# Autodesk Inventor assembly: Prototype2
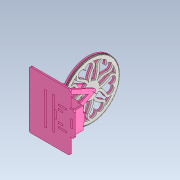
[picture p0: Inventor's stored thumbnail of the model, 180x180]
Saved by Autodesk Inventor 2021 (Build 250183000, 183)
## iProperties
Created: 2021-08-31
Part Number: Prototype2
Document SubType Name: Assembly
Designer: digge
Author: digge
## Documents named in this file (11)
- C:\Users\digge\Documents\Inventor\Projects\FerrisWheel\Prototype2.iam
- C:\Users\digge\Documents\Inventor\Projects\FerrisWheel\Base.ipt
- C:\Users\digge\Documents\Inventor\Projects\FerrisWheel\SideWall.ipt
- C:\Users\digge\Documents\Inventor\Projects\FerrisWheel\FrontWall.ipt
- C:\Users\digge\Documents\Inventor\Projects\FerrisWheel\BackWall.ipt
- C:\Users\digge\Documents\Inventor\Projects\FerrisWheel\Stand.ipt
- C:\Users\digge\Documents\Inventor\Projects\FerrisWheel\Screw.ipt
- C:\Users\digge\Documents\Inventor\Projects\FerrisWheel\WheelFace.ipt
- C:\Users\digge\Documents\Inventor\Projects\FerrisWheel\WheelGear.iam
- C:\Users\digge\Documents\Inventor\Projects\FerrisWheel\MotorGear.iam
- C:\Users\digge\Documents\Inventor\Projects\FerrisWheel\Motor.ipt
## Components (12 placed, 10 different names)
1. Base:1 — Flush:1, Flush:2, Mate:1, Mate:2, Mate:3, Mate:4, Flush:3, Mate:5, Mate:6, Flush:4, Mate:7, Mate:8, Flush:5, Flush:6, Mate:9, Mate:10, Mate:11, Mate:12
2. SideWall:1 — Flush:1, Mate:1, Mate:2
3. SideWall:2 — Flush:2, Mate:3, Mate:4
4. FrontWall:1 — Flush:4, Mate:7, Mate:8
5. BackWall:1 — Flush:3, Mate:5, Mate:6, Mate:17
6. Stand:1 — Flush:5, Mate:11, Mate:12, Mate:15
7. Stand:2 — Flush:6, Mate:9, Mate:10, Insert:1
8. Screw:1 — Insert:1, Mate:13, Mate:14
9. WheelFace:1 — Mate:13, Mate:16, Rotation:1, Mate:18
10. WheelGear:1 [sub-assembly] — Mate:14, Mate:15, Mate:16, Rotation:1
11. Motor:1 — Mate:17
12. MotorGear:1 [sub-assembly] — Mate:18
## Relationships (26: Mate 18, Flush 6, Insert 1, RelateRotation 1)
- Flush:1: Base:1 ↔ SideWall:1
- Flush:2: Base:1 ↔ SideWall:2
- Mate:1: Base:1 ↔ SideWall:1
- Mate:2: Base:1 ↔ SideWall:1
- Mate:3: Base:1 ↔ SideWall:2
- Mate:4: Base:1 ↔ SideWall:2
- Flush:3: Base:1 ↔ BackWall:1
- Mate:5: Base:1 ↔ BackWall:1
- Mate:6: Base:1 ↔ BackWall:1
- Flush:4: Base:1 ↔ FrontWall:1
- Mate:7: Base:1 ↔ FrontWall:1
- Mate:8: Base:1 ↔ FrontWall:1
- Flush:5: Base:1 ↔ Stand:1
- Flush:6: Base:1 ↔ Stand:2
- Mate:9: Base:1 ↔ Stand:2
- Mate:10: Base:1 ↔ Stand:2
- Mate:11: Base:1 ↔ Stand:1
- Mate:12: Base:1 ↔ Stand:1
- Insert:1: Stand:2 ↔ Screw:1
- Mate:13: Screw:1 ↔ WheelFace:1
- Mate:14: Screw:1 ↔ WheelGear:1
- Mate:15: Stand:1 ↔ WheelGear:1
- Mate:16: WheelFace:1 ↔ WheelGear:1
- Rotation:1 [RelateRotation] (1 ul): WheelFace:1 ↔ WheelGear:1
- Mate:17: BackWall:1 ↔ Motor:1
- Mate:18: WheelFace:1 ↔ MotorGear:1
